# Autodesk Inventor assembly: Füllstandsmessung
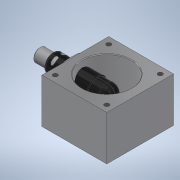
[picture p0: Inventor's stored thumbnail of the model, 180x180]
Saved by Autodesk Inventor 2021 (Build 250183000, 183)
## iProperties
Created: 2021-04-27
Part Number: Füllstandsmessung
Material: Generisch
Document SubType Name: Assembly
Designer: Michael
Author: Michael
## Documents named in this file (5)
- C:\Users\Sebastian Seewald\Documents\Inventor\Konstruktion_Studium\Lernfabrik\104_Extrudereinheit\204.001.01_ZB_Sensor_Aufnahme.iam
- C:\Users\Sebastian Seewald\Documents\Inventor\Konstruktion_Studium\Lernfabrik\104_Extrudereinheit\104.001.01_Sensoraufnahme.ipt
- C:\Users\Sebastian Seewald\Documents\Inventor\Konstruktion_Studium\Lernfabrik\104_Extrudereinheit\504.001.01_BALLUFF-BUS-W18M1-XA-07_035-S92G_01.ipt
- C:\Users\Sebastian Seewald\Documents\Inventor\Konstruktion_Studium\Lernfabrik\104_Extrudereinheit\504.002.01_BALLUFF-BUS-W18M1-XA-07_035-S92G_Mutter.ipt
- C:\Users\Sebastian Seewald\Documents\Inventor\Konstruktion_Studium\Lernfabrik\104_Extrudereinheit\504.004.01_O-Ring_ID50_AD54.ipt
## Components (4 placed, 4 different names)
1. 104.001.01_Sensoraufnahme:1 — Passend:5, Passend:8, Winkel:1, Passend:9, Fluchtend:1, Passend:10, Winkel:2, Passend:15, Passend:16
2. 504.001.01_BALLUFF-BUS-W18M1-XA-07_035-S92G_01:2 — Passend:5, Passend:7, Winkel:1, Passend:10
3. 504.002.01_BALLUFF-BUS-W18M1-XA-07_035-S92G_Mutter:2 — Passend:7, Passend:8
4. 504.004.01_O-Ring_ID50_AD54:1 — Passend:15, Passend:16
## Relationships (10: Mate 7, Angle 2, Flush 1)
- Passend:5 [Mate]: 104.001.01_Sensoraufnahme:1 ↔ 504.001.01_BALLUFF-BUS-W18M1-XA-07_035-S92G_01:2
- Passend:7 [Mate]: 504.001.01_BALLUFF-BUS-W18M1-XA-07_035-S92G_01:2 ↔ 504.002.01_BALLUFF-BUS-W18M1-XA-07_035-S92G_Mutter:2
- Passend:8 [Mate]: 104.001.01_Sensoraufnahme:1 ↔ 504.002.01_BALLUFF-BUS-W18M1-XA-07_035-S92G_Mutter:2
- Winkel:1 [Angle] (-90 deg): 104.001.01_Sensoraufnahme:1 ↔ 504.001.01_BALLUFF-BUS-W18M1-XA-07_035-S92G_01:2
- Passend:9 [Mate]: 104.001.01_Sensoraufnahme:1
- Fluchtend:1 [Flush]: 104.001.01_Sensoraufnahme:1
- Passend:10 [Mate]: 104.001.01_Sensoraufnahme:1 ↔ 504.001.01_BALLUFF-BUS-W18M1-XA-07_035-S92G_01:2
- Winkel:2 [Angle] (0 deg): 104.001.01_Sensoraufnahme:1
- Passend:15 [Mate]: 104.001.01_Sensoraufnahme:1 ↔ 504.004.01_O-Ring_ID50_AD54:1
- Passend:16 [Mate] (-6 mm): 104.001.01_Sensoraufnahme:1 ↔ 504.004.01_O-Ring_ID50_AD54:1
